# Autodesk Inventor assembly: Final Body
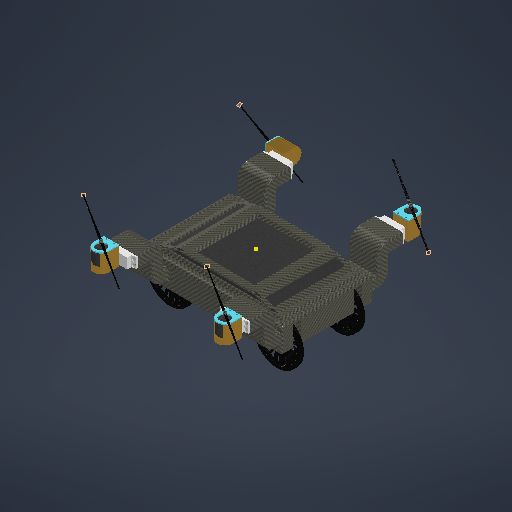
[picture p0: Inventor's stored thumbnail of the model, 512x512]
Saved by Autodesk Inventor 2026.1 (Build 301233000, 233)
## iProperties
Created: 2026-07-11
Part Number: Final Body
Document SubType Name: Assembly
Designer: ankit
Author: ankit
## Documents named in this file (11)
- C:\Users\ankit\OneDrive\Documents\Personal\3D designs\3D Printing Model\Major project\With Servo\Final Body.iam
- C:\Users\ankit\OneDrive\Documents\Personal\3D designs\3D Printing Model\Major project\With Servo\Body.ipt
- C:\Users\ankit\OneDrive\Documents\Personal\3D designs\3D Printing Model\Major project\With Servo\Servo.ipt
- C:\Users\ankit\OneDrive\Documents\Personal\3D designs\3D Printing Model\Major project\With Servo\BLDC Holder.ipt
- C:\Users\ankit\OneDrive\Documents\Personal\3D designs\3D Printing Model\Major project\With Servo\Bearing.ipt
- C:\Users\ankit\OneDrive\Documents\Personal\3D designs\3D Printing Model\Major project\With Servo\Motor.ipt
- C:\Users\ankit\OneDrive\Documents\Personal\3D designs\3D Printing Model\Major project\With Servo\Propeller.ipt
- C:\Users\ankit\OneDrive\Documents\Personal\3D designs\3D Printing Model\Major project\With Servo\Connecting Rod.ipt
- C:\Users\ankit\OneDrive\Documents\Personal\3D designs\3D Printing Model\Major project\With Servo\Tyres.ipt
- C:\Users\ankit\OneDrive\Documents\Personal\3D designs\3D Printing Model\Major project\With Servo\Top Cover.ipt
- C:\Users\ankit\OneDrive\Documents\Personal\3D designs\3D Printing Model\Major project\With Servo\Holder Cover.ipt
## Components (38 placed, 10 different names)
1. Body:1 — Rigid:1, Rigid:2, Rigid:3, Rigid:4, Rigid:9, Rigid:10, Rigid:11, Rigid:12, Rigid:13, Rigid:14, Rigid:15, Rigid:16, Rigid:33
2. Servo:1 — Rigid:1, Rigid:7
3. Servo:2 — Rigid:2, Rigid:8
4. Servo:3 — Rigid:3, Rigid:5
5. Servo:4 — Rigid:4, Rigid:6
6. BLDC Holder:1 — Rigid:5, Rigid:18, Rigid:36
7. BLDC Holder:2 — Rigid:6, Rigid:19, Rigid:35
8. BLDC Holder:3 — Rigid:7, Rigid:17, Rigid:34
9. BLDC Holder:4 — Rigid:8, Rigid:20, Rigid:37
10. Bearing:1 — Rigid:12
11. Bearing:2 — Rigid:11, Rigid:25
12. Bearing:3 — Rigid:15, Rigid:27
13. Bearing:4 — Rigid:14
14. Bearing:5 — Rigid:10, Rigid:26
15. Bearing:6 — Rigid:9
16. Bearing:7 — Rigid:13, Rigid:28
17. Bearing:8 — Rigid:16
18. Motor:1 — Rigid:19, Rigid:23
19. Motor:2 — Rigid:20, Rigid:22
20. Motor:3 — Rigid:18, Rigid:24
21. Motor:4 — Rigid:17, Rigid:21
22. Propeller:1 — Rigid:22
23. Propeller:2 — Rigid:21
24. Propeller:3 — Rigid:23
25. Propeller:4 — Rigid:24
26. Connecting Rod:1 — Rigid:27, Rigid:30
27. Connecting Rod:2 — Rigid:26, Rigid:29
28. Connecting Rod:3 — Rigid:25, Rigid:32
29. Connecting Rod:4 — Rigid:28, Rigid:31
30. Tyres:1 — Rigid:32
31. Tyres:2 — Rigid:31
32. Tyres:3 — Rigid:29
33. Tyres:4 — Rigid:30
34. Top Cover:1 — Rigid:33
35. Holder Cover:1 — Rigid:37
36. Holder Cover:2 — Rigid:34
37. Holder Cover:3 — Rigid:35
38. Holder Cover:4 — Rigid:36
## Relationships (37: WeldJoint 37)
- Rigid:1 [WeldJoint]: Body:1 ↔ Servo:1
- Rigid:2 [WeldJoint]: Body:1 ↔ Servo:2
- Rigid:3 [WeldJoint]: Body:1 ↔ Servo:3
- Rigid:4 [WeldJoint]: Body:1 ↔ Servo:4
- Rigid:5 [WeldJoint]: Servo:3 ↔ BLDC Holder:1
- Rigid:6 [WeldJoint]: Servo:4 ↔ BLDC Holder:2
- Rigid:7 [WeldJoint]: Servo:1 ↔ BLDC Holder:3
- Rigid:8 [WeldJoint]: Servo:2 ↔ BLDC Holder:4
- Rigid:9 [WeldJoint]: Body:1 ↔ Bearing:6
- Rigid:10 [WeldJoint]: Body:1 ↔ Bearing:5
- Rigid:11 [WeldJoint]: Body:1 ↔ Bearing:2
- Rigid:12 [WeldJoint]: Body:1 ↔ Bearing:1
- Rigid:13 [WeldJoint]: Body:1 ↔ Bearing:7
- Rigid:14 [WeldJoint]: Body:1 ↔ Bearing:4
- Rigid:15 [WeldJoint]: Body:1 ↔ Bearing:3
- Rigid:16 [WeldJoint]: Body:1 ↔ Bearing:8
- Rigid:17 [WeldJoint]: BLDC Holder:3 ↔ Motor:4
- Rigid:18 [WeldJoint]: BLDC Holder:1 ↔ Motor:3
- Rigid:19 [WeldJoint]: BLDC Holder:2 ↔ Motor:1
- Rigid:20 [WeldJoint]: BLDC Holder:4 ↔ Motor:2
- Rigid:21 [WeldJoint]: Motor:4 ↔ Propeller:2
- Rigid:22 [WeldJoint]: Motor:2 ↔ Propeller:1
- Rigid:23 [WeldJoint]: Motor:1 ↔ Propeller:3
- Rigid:24 [WeldJoint]: Motor:3 ↔ Propeller:4
- Rigid:25 [WeldJoint] (5 mm): Bearing:2 ↔ Connecting Rod:3
- Rigid:26 [WeldJoint] (5 mm): Bearing:5 ↔ Connecting Rod:2
- Rigid:27 [WeldJoint] (5 mm): Bearing:3 ↔ Connecting Rod:1
- Rigid:28 [WeldJoint] (5 mm): Bearing:7 ↔ Connecting Rod:4
- Rigid:29 [WeldJoint] (4 mm): Connecting Rod:2 ↔ Tyres:3
- Rigid:30 [WeldJoint] (-4 mm): Connecting Rod:1 ↔ Tyres:4
- Rigid:31 [WeldJoint] (-4 mm): Connecting Rod:4 ↔ Tyres:2
- Rigid:32 [WeldJoint] (4 mm): Connecting Rod:3 ↔ Tyres:1
- Rigid:33 [WeldJoint]: Body:1 ↔ Top Cover:1
- Rigid:34 [WeldJoint] (-2 mm): BLDC Holder:3 ↔ Holder Cover:2
- Rigid:35 [WeldJoint]: BLDC Holder:2 ↔ Holder Cover:3
- Rigid:36 [WeldJoint]: BLDC Holder:1 ↔ Holder Cover:4
- Rigid:37 [WeldJoint]: BLDC Holder:4 ↔ Holder Cover:1
